# Autodesk Inventor assembly: ArmBaseAssembly
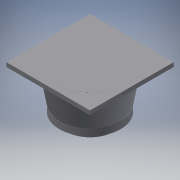
[picture p0: Inventor's stored thumbnail of the model, 180x180]
Saved by Autodesk Inventor 2019 (Build 230136000, 136)
## iProperties
Created: 2021-05-14
Part Number: ArmBaseAssembly
Document SubType Name: Assembly
Designer: Eric
Author: Eric
## Documents named in this file (5)
- C:\Users\Eric\Documents\! - Uni\Year 4\MENG-Robot-Fab-Project\Models\For_Optimiser\Static Parts Assembly\Arm base assembly\ArmBaseAssembly.iam
- C:\Users\Eric\Documents\! - Uni\Year 4\MENG-Robot-Fab-Project\Denavit-Hartneberg Tests\Models\ArmSegments\ArmBase_topRing.ipt
- C:\Users\Eric\Documents\! - Uni\Year 4\MENG-Robot-Fab-Project\Denavit-Hartneberg Tests\Models\ArmSegments\ArmBase_bottomRing.ipt
- C:\Users\Eric\Documents\! - Uni\Year 4\MENG-Robot-Fab-Project\Denavit-Hartneberg Tests\Models\ArmSegments\ArmBase_frustum.ipt
- C:\Users\Eric\Documents\! - Uni\Year 4\MENG-Robot-Fab-Project\Denavit-Hartneberg Tests\Models\ArmSegments\ArmBase_basePlate.ipt
## Components (4 placed, 4 different names)
1. ArmBase_topRing:1 — Flush:1, Mate:1
2. ArmBase_bottomRing:1
3. ArmBase_frustum:1 — Flush:1
4. ArmBase_basePlate:1
## Relationships (2: Flush 1, Mate 1)
- Flush:1: ArmBase_topRing:1 ↔ ArmBase_frustum:1
- Mate:1: ArmBase_topRing:1
